# Autodesk Inventor assembly: NGC Assembly
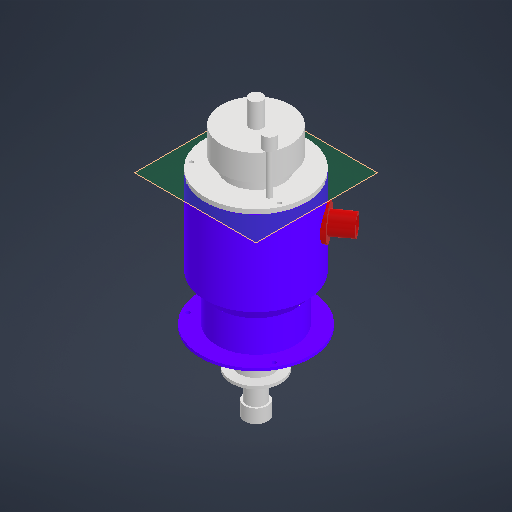
[picture p0: Inventor's stored thumbnail of the model, 512x512]
Saved by Autodesk Inventor 2026 (Build 300175050, 175E)
## iProperties
Created: 2025-07-02
Part Number: NGC Assembly
Document SubType Name: Assembly
Designer: user
Author: user
## Documents named in this file (3)
- C:\Projects\CryocoolerHybrid98\NGC Assembly.iam
- C:\Projects\CryocoolerHybrid98\STI NGC Cooling Shroud.ipt
- C:\Projects\CryocoolerHybrid98\STI NGC Cryocooler.ipt
## Components (2 placed, 2 different names)
1. STI NGC Cooling Shroud:1 — Flush:1, Flush:2, Flush:3, Mate:1, Mate:2, Mate:3, Mate:4, Mate:5, Mate:6, Mate:7, Mate:8
2. STI NGC Cryocooler:1 — Mate:5, Mate:6, Mate:7, Mate:8
## Relationships (11: Mate 8, Flush 3)
- Flush:1: STI NGC Cooling Shroud:1
- Flush:2: STI NGC Cooling Shroud:1
- Flush:3: STI NGC Cooling Shroud:1
- Mate:1: STI NGC Cooling Shroud:1
- Mate:2: STI NGC Cooling Shroud:1
- Mate:3: STI NGC Cooling Shroud:1
- Mate:4: STI NGC Cooling Shroud:1
- Mate:5: STI NGC Cooling Shroud:1 ↔ STI NGC Cryocooler:1
- Mate:6: STI NGC Cooling Shroud:1 ↔ STI NGC Cryocooler:1
- Mate:7: STI NGC Cooling Shroud:1 ↔ STI NGC Cryocooler:1
- Mate:8: STI NGC Cooling Shroud:1 ↔ STI NGC Cryocooler:1
